# Autodesk Inventor assembly: fridge
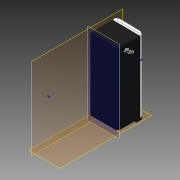
[picture p0: Inventor's stored thumbnail of the model, 180x180]
Saved by Autodesk Inventor 2015 (Build 190159000, 159)
## iProperties
Created: 2015-10-19
Part Number: fridge
Document SubType Name: Assembly
Designer: omae
Author: omae
## Documents named in this file (2)
- C:\Users\omae\Desktop\研究室\論文・資料\ROS\kitchen\stl\fridge.iam
- C:\Users\omae\Desktop\研究室\論文・資料\ROS\kitchen\toolinstall\HELADERA1\HELADERA1.iam
## Components (1 placed, 1 different names)
1. HELADERA1:1 [sub-assembly] — メイト:1, メイト:2, メイト:3
## Relationships (3: Mate 3)
- メイト:1 [Mate]: HELADERA1:1
- メイト:2 [Mate]: HELADERA1:1
- メイト:3 [Mate]: HELADERA1:1
